# Autodesk Inventor assembly: mini-vessel
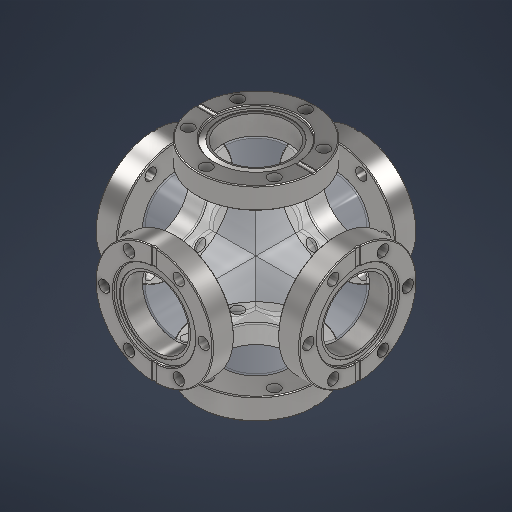
[picture p0: Inventor's stored thumbnail of the model, 512x512]
Saved by Autodesk Inventor 2026 (Build 300175050, 175E)
## iProperties
Created: 2025-07-13
Part Number: mini-vessel
Document SubType Name: Assembly
Designer: jin20
Author: jin20
## Documents named in this file (3)
- C:\Users\jin20\Documents\装置CAD\RamanSystem\vessel\mini-vessel.iam
- C:\Users\jin20\Documents\装置CAD\PIHTI\ContentCenter\CF-parts\CF70-nipple\cf70_hole_nipple.ipt
- C:\Users\jin20\Documents\装置CAD\RamanSystem\vessel\mini-vessel_base.ipt
## Components (7 placed, 2 different names)
1. cf70_hole_nipple:1 — 挿入:6
2. cf70_hole_nipple:2 — 挿入:2
3. cf70_hole_nipple:3 — 挿入:3
4. cf70_hole_nipple:4 — 挿入:5
5. cf70_hole_nipple:5 — 挿入:4
6. cf70_hole_nipple:6 — 挿入:1
7. mini-vessel_base:1 — 挿入:1, 挿入:2, 挿入:3, 挿入:4, 挿入:5, 挿入:6
## Relationships (6: Insert 6)
- 挿入:1 [Insert]: cf70_hole_nipple:6 ↔ mini-vessel_base:1
- 挿入:2 [Insert]: cf70_hole_nipple:2 ↔ mini-vessel_base:1
- 挿入:3 [Insert]: cf70_hole_nipple:3 ↔ mini-vessel_base:1
- 挿入:4 [Insert]: cf70_hole_nipple:5 ↔ mini-vessel_base:1
- 挿入:5 [Insert]: cf70_hole_nipple:4 ↔ mini-vessel_base:1
- 挿入:6 [Insert]: cf70_hole_nipple:1 ↔ mini-vessel_base:1
